# Autodesk Inventor assembly: Kinect
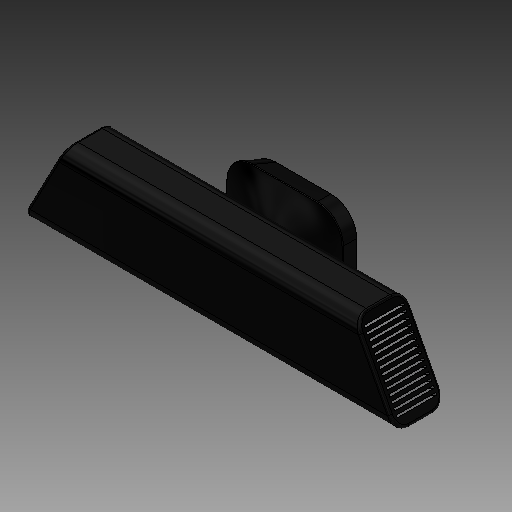
[picture p0: Inventor's stored thumbnail of the model, 512x512]
Saved by Autodesk Inventor 2018 (Build 220112000, 112)
## iProperties
Created: 2012-12-04
Part Number: Kinect
Document SubType Name: Assembly
Designer: AYUSH SHUKLA
Sending System: SolidWorks 2012
Last Author: Andy
Last Saved: 2012-12-12
Author: AYUSH SHUKLA
## Documents named in this file (3)
- C:\Study\BTP2\Robomuse Inventor CAD\kinect\Kinect.iam
- C:\Study\BTP2\Robomuse Inventor CAD\Kinect\base.ipt
- C:\Study\BTP2\Robomuse Inventor CAD\Kinect\kinect_body.ipt
## Components (2 placed, 2 different names)
1. base KINECT:1 — Ball:1, Angle:1, Angle:2
2. KINECT XBOX:1 — Ball:1, Angle:1, Angle:2
## Relationships (3: Angle 2, BallJoint 1)
- Ball:1: base KINECT:1 ↔ KINECT XBOX:1
- Angle:1 (180 deg): base KINECT:1 ↔ KINECT XBOX:1
- Angle:2 (0 deg): base KINECT:1 ↔ KINECT XBOX:1
